# Autodesk Inventor assembly: Assembly 2
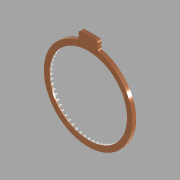
[picture p0: Inventor's stored thumbnail of the model, 180x180]
Saved by Autodesk Inventor 2020 (Build 240168000, 168)
## iProperties
Created: 2020-10-17
Part Number: Assembly 2
Document SubType Name: Assembly
Designer: user
Author: user
## Documents named in this file (5)
- D:\Documents\Github\Arduino-Smart-light\3DModel\Wall\Assembly CNC.iam
- C:\Users\user\Google Drive\Projects\3d\4 Projects\AA Done\.Parts\WS2812B\WS2812B Black 60leds_m v7.iam
- D:\Documents\Github\Arduino-Smart-light\3DModel\Wall\PCB.ipt
- C:\Users\user\Google Drive\Projects\3d\4 Projects\AA Done\.Parts\ESP32.ipt
- D:\Documents\Github\Arduino-Smart-light\3DModel\Wall\Wall Clock CNC.ipt
## Components (63 placed, 4 different names)
1. Wall Clock CNC:1 — Angle:2, Mate:7, Mate:8, Flush:3, Mate:10, Mate:11, Mate:12, Flush:6
2. PCB:1 — Mate:9, Flush:4, Flush:5
3. ESP32:1 — Flush:3, Mate:9, Flush:4, Flush:5, Mate:10, Mate:11
4. WS2812B Black 60leds_m v7:61 [sub-assembly] — Angle:2, Mate:7, Mate:8
5. WS2812B Black 60leds_m v7:62 [sub-assembly]
6. WS2812B Black 60leds_m v7:63 [sub-assembly]
7. WS2812B Black 60leds_m v7:64 [sub-assembly]
8. WS2812B Black 60leds_m v7:65 [sub-assembly]
9. WS2812B Black 60leds_m v7:66 [sub-assembly]
10. WS2812B Black 60leds_m v7:67 [sub-assembly]
11. WS2812B Black 60leds_m v7:68 [sub-assembly]
12. WS2812B Black 60leds_m v7:69 [sub-assembly]
13. WS2812B Black 60leds_m v7:70 [sub-assembly]
14. WS2812B Black 60leds_m v7:71 [sub-assembly]
15. WS2812B Black 60leds_m v7:72 [sub-assembly]
16. WS2812B Black 60leds_m v7:73 [sub-assembly]
17. WS2812B Black 60leds_m v7:74 [sub-assembly]
18. WS2812B Black 60leds_m v7:75 [sub-assembly]
19. WS2812B Black 60leds_m v7:76 [sub-assembly]
20. WS2812B Black 60leds_m v7:77 [sub-assembly]
21. WS2812B Black 60leds_m v7:78 [sub-assembly]
22. WS2812B Black 60leds_m v7:79 [sub-assembly]
23. WS2812B Black 60leds_m v7:80 [sub-assembly]
24. WS2812B Black 60leds_m v7:81 [sub-assembly]
25. WS2812B Black 60leds_m v7:82 [sub-assembly]
26. WS2812B Black 60leds_m v7:83 [sub-assembly]
27. WS2812B Black 60leds_m v7:84 [sub-assembly]
28. WS2812B Black 60leds_m v7:85 [sub-assembly]
29. WS2812B Black 60leds_m v7:86 [sub-assembly]
30. WS2812B Black 60leds_m v7:87 [sub-assembly]
31. WS2812B Black 60leds_m v7:88 [sub-assembly]
32. WS2812B Black 60leds_m v7:89 [sub-assembly]
33. WS2812B Black 60leds_m v7:90 [sub-assembly]
34. WS2812B Black 60leds_m v7:91 [sub-assembly]
35. WS2812B Black 60leds_m v7:92 [sub-assembly]
36. WS2812B Black 60leds_m v7:93 [sub-assembly]
37. WS2812B Black 60leds_m v7:94 [sub-assembly]
38. WS2812B Black 60leds_m v7:95 [sub-assembly]
39. WS2812B Black 60leds_m v7:96 [sub-assembly]
40. WS2812B Black 60leds_m v7:97 [sub-assembly]
41. WS2812B Black 60leds_m v7:98 [sub-assembly]
42. WS2812B Black 60leds_m v7:99 [sub-assembly]
43. WS2812B Black 60leds_m v7:100 [sub-assembly]
44. WS2812B Black 60leds_m v7:101 [sub-assembly]
45. WS2812B Black 60leds_m v7:102 [sub-assembly]
46. WS2812B Black 60leds_m v7:103 [sub-assembly]
47. WS2812B Black 60leds_m v7:104 [sub-assembly]
48. WS2812B Black 60leds_m v7:105 [sub-assembly]
49. WS2812B Black 60leds_m v7:106 [sub-assembly]
50. WS2812B Black 60leds_m v7:107 [sub-assembly]
51. WS2812B Black 60leds_m v7:108 [sub-assembly]
52. WS2812B Black 60leds_m v7:109 [sub-assembly]
53. WS2812B Black 60leds_m v7:110 [sub-assembly]
54. WS2812B Black 60leds_m v7:111 [sub-assembly]
55. WS2812B Black 60leds_m v7:112 [sub-assembly]
56. WS2812B Black 60leds_m v7:113 [sub-assembly]
57. WS2812B Black 60leds_m v7:114 [sub-assembly]
58. WS2812B Black 60leds_m v7:115 [sub-assembly]
59. WS2812B Black 60leds_m v7:116 [sub-assembly]
60. WS2812B Black 60leds_m v7:117 [sub-assembly]
61. WS2812B Black 60leds_m v7:118 [sub-assembly]
62. WS2812B Black 60leds_m v7:119 [sub-assembly]
63. WS2812B Black 60leds_m v7:120 [sub-assembly]
## Component patterns: LEDs (60 elements)
## Relationships (11: Mate 6, Flush 4, Angle 1)
- Angle:2 (0 deg): Wall Clock CNC:1 ↔ WS2812B Black 60leds_m v7:61
- Mate:7: Wall Clock CNC:1 ↔ WS2812B Black 60leds_m v7:61
- Mate:8 (18.367 mm): Wall Clock CNC:1 ↔ WS2812B Black 60leds_m v7:61
- Flush:3: Wall Clock CNC:1 ↔ ESP32:1
- Mate:9 (0.5 mm): PCB:1 ↔ ESP32:1
- Flush:4: PCB:1 ↔ ESP32:1
- Flush:5: PCB:1 ↔ ESP32:1
- Mate:10 (0.2 mm): Wall Clock CNC:1 ↔ ESP32:1
- Mate:11 (0.2 mm): Wall Clock CNC:1 ↔ ESP32:1
- Mate:12: Wall Clock CNC:1
- Flush:6: Wall Clock CNC:1
